# Autodesk Inventor assembly: Frame Assembly
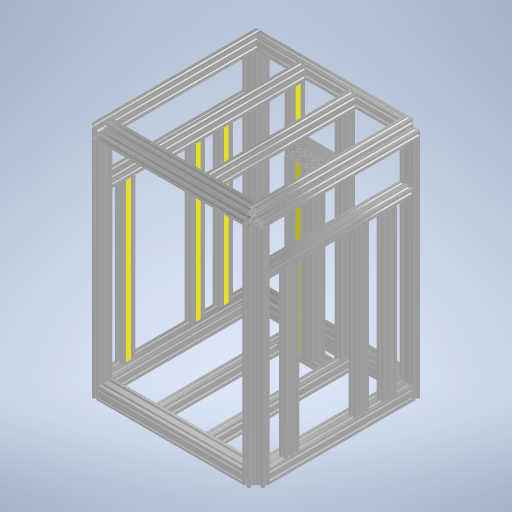
[picture p0: Inventor's stored thumbnail of the model, 512x512]
Saved by Autodesk Inventor 2024 (Build 280153000, 153)
## iProperties
Created: 2024-12-10
Part Number: Frame Assembly
Document SubType Name: Assembly
Designer: Ishaan
Author: Ishaan
## Documents named in this file (27)
- E:\Projects\Axiom--IDEX-3D-Printer\CAD\01 - Frame\Frame Assembly.iam
- E:\Projects\Axiom--IDEX-3D-Printer\CAD\01 - Frame\4040 Back Left Corner.ipt
- E:\Projects\Axiom--IDEX-3D-Printer\CAD\01 - Frame\4040 Back Right Corner.ipt
- E:\Projects\Axiom--IDEX-3D-Printer\CAD\01 - Frame\4040 Front Left Corner.ipt
- E:\Projects\Axiom--IDEX-3D-Printer\CAD\01 - Frame\4040 Front Right Corner.ipt
- E:\Projects\Axiom--IDEX-3D-Printer\CAD\01 - Frame\Front Base Beam.ipt
- E:\Projects\Axiom--IDEX-3D-Printer\CAD\01 - Frame\Left Base Beam.ipt
- E:\Projects\Axiom--IDEX-3D-Printer\CAD\01 - Frame\Rear Base Beam.ipt
- E:\Projects\Axiom--IDEX-3D-Printer\CAD\01 - Frame\Right Base Beam.ipt
- E:\Projects\Axiom--IDEX-3D-Printer\CAD\01 - Frame\2040 Side Anterior Riser.ipt
- E:\Projects\Axiom--IDEX-3D-Printer\CAD\01 - Frame\2040 Side Posterior Riser.ipt
- E:\Projects\Axiom--IDEX-3D-Printer\CAD\01 - Frame\2040 Side Medial Riser.ipt
- E:\Projects\Axiom--IDEX-3D-Printer\CAD\01 - Frame\2040 Left Gantry Extrusion.ipt
- E:\Projects\Axiom--IDEX-3D-Printer\CAD\01 - Frame\2040 Right Gantry Extrusion.ipt
- E:\Projects\Axiom--IDEX-3D-Printer\CAD\01 - Frame\2040 Bottom Left Reinforcement.ipt
- E:\Projects\Axiom--IDEX-3D-Printer\CAD\01 - Frame\2040 Bottom Right Reinforcement.ipt
- E:\Projects\Axiom--IDEX-3D-Printer\CAD\01 - Frame\4040 Top Left Edge.ipt
- E:\Projects\Axiom--IDEX-3D-Printer\CAD\01 - Frame\4040 Top Right Edge.ipt
- E:\Projects\Axiom--IDEX-3D-Printer\CAD\01 - Frame\4040 Top Front Edge.ipt
- E:\Projects\Axiom--IDEX-3D-Printer\CAD\01 - Frame\4040 Top Rear Edge.ipt
- E:\Projects\Axiom--IDEX-3D-Printer\CAD\01 - Frame\2040 Top Left Reinforcement.ipt
- E:\Projects\Axiom--IDEX-3D-Printer\CAD\01 - Frame\2040 Top Right Reinforcement.ipt
- E:\Projects\Axiom--IDEX-3D-Printer\CAD\01 - Frame\2040 Rear Left Riser.ipt
- E:\Projects\Axiom--IDEX-3D-Printer\CAD\01 - Frame\2040 Rear Right Riser.ipt
- E:\Projects\Axiom--IDEX-3D-Printer\CAD\01 - Frame\2040 Z-Rail Brace.ipt
- E:\Projects\Axiom--IDEX-3D-Printer\CAD\01 - Frame\2040 Z-column Support.ipt
- E:\Projects\Axiom--IDEX-3D-Printer\CAD\01 - Frame\4080 Z-rail.ipt
## Components (29 placed, 26 different names)
1. 4040 Back Left Corner:1 — Flush:11, Mate:7, Flush:12, Mate:9, Flush:14, Mate:17
2. 4040 Back Right Corner:1 — Flush:3, Mate:3, Flush:4, Mate:8, Mate:15
3. 4040 Front Left Corner:1 — Flush:7, Mate:5, Flush:8, Mate:6, Flush:9, Flush:10, Flush:16, Mate:13, Mate:23, Mate:30, Flush:25, Flush:26
4. 4040 Front Right Corner:1 — Flush:1, Mate:2, Flush:2, Mate:4, Flush:6, Mate:11, Mate:25, Flush:27, Mate:31, Flush:28
5. Front Base Beam:1 — Flush:5, Mate:4, Flush:6, Flush:7, Mate:5, Flush:8, Mate:26, Flush:23, Mate:28, Flush:24
6. Left Base Beam:1 — Mate:6, Flush:9, Flush:10, Flush:11, Mate:7, Flush:12, Mate:12, Flush:18, Mate:16, Mate:20, Flush:20, Mate:27
7. Rear Base Beam:1 — Flush:13, Mate:8, Mate:9, Flush:14
8. Right Base Beam:1 — Mate:1, Flush:1, Mate:2, Flush:2, Flush:3, Mate:3, Flush:4, Flush:5, Flush:13, Mate:10, Flush:15, Mate:14, Flush:17, Mate:18, Flush:19, Mate:29
9. 2040 Side Anterior Riser:1 — Mate:10, Flush:15, Mate:11, Mate:19, Flush:22
10. 2040 Side Anterior Riser:2 — Mate:12, Flush:16, Mate:13, Mate:21
11. 2040 Side Posterior Riser:1 — Mate:14, Flush:17, Mate:15, Mate:24, Mate:43
12. 2040 Side Posterior Riser:2 — Flush:18, Mate:16, Mate:17, Flush:42
13. 2040 Side Medial Riser:1 — Mate:18, Flush:19, Mate:19
14. 2040 Side Medial Riser:2 — Mate:20, Flush:20, Mate:21, Mate:22, Flush:21
15. 2040 Left Gantry Extrusion:1 — Mate:22, Mate:23, Flush:21
16. 2040 Right Gantry Extrusion:1 — Mate:24, Mate:25, Flush:22
17. 2040 Bottom Left Reinforcement:1 — Mate:28, Flush:24, Mate:29, Mate:40, Flush:33, Mate:48
18. 2040 Bottom Right Reinforcement:1 — Mate:26, Flush:23, Mate:27, Mate:42, Flush:34, Flush:41
19. 4040 Top Left Edge:1 — Flush:27, Mate:31, Flush:28, Mate:39
20. 4040 Top Right Edge:1 — Mate:30, Flush:25, Flush:26, Mate:37
21. 4040 Top Rear Edge:1
22. 4040 Top Front Edge:2 — Mate:36, Flush:31, Mate:38, Flush:32
23. 2040 Top Left Reinforcement:1 — Mate:38, Flush:32, Mate:39
24. 2040 Top Right Reinforcement:1 — Mate:36, Flush:31, Mate:37
25. 2040 Rear Left Riser:1 — Mate:42, Flush:34, Flush:35, Mate:47, Flush:40, Mate:50
26. 2040 Rear Right Riser:1 — Mate:40, Flush:33, Flush:35, Mate:43
27. 2040 Z-Rail Brace:1 — Mate:47, Flush:40, Flush:44
28. 2040 Z-column Support:1 — Flush:41, Mate:48, Flush:42, Mate:49, Flush:43
29. 4080 Z-rail:1 — Mate:49, Flush:43, Mate:50, Flush:44
## Relationships (86: Mate 46, Flush 40)
- Mate:1: Right Base Beam:1
- Flush:1: 4040 Front Right Corner:1 ↔ Right Base Beam:1
- Mate:2: 4040 Front Right Corner:1 ↔ Right Base Beam:1
- Flush:2: 4040 Front Right Corner:1 ↔ Right Base Beam:1
- Flush:3: 4040 Back Right Corner:1 ↔ Right Base Beam:1
- Mate:3: 4040 Back Right Corner:1 ↔ Right Base Beam:1
- Flush:4: 4040 Back Right Corner:1 ↔ Right Base Beam:1
- Flush:5: Front Base Beam:1 ↔ Right Base Beam:1
- Mate:4: 4040 Front Right Corner:1 ↔ Front Base Beam:1
- Flush:6: 4040 Front Right Corner:1 ↔ Front Base Beam:1
- Flush:7: 4040 Front Left Corner:1 ↔ Front Base Beam:1
- Mate:5: 4040 Front Left Corner:1 ↔ Front Base Beam:1
- Flush:8: 4040 Front Left Corner:1 ↔ Front Base Beam:1
- Mate:6: 4040 Front Left Corner:1 ↔ Left Base Beam:1
- Flush:9: 4040 Front Left Corner:1 ↔ Left Base Beam:1
- Flush:10: 4040 Front Left Corner:1 ↔ Left Base Beam:1
- Flush:11: 4040 Back Left Corner:1 ↔ Left Base Beam:1
- Mate:7: 4040 Back Left Corner:1 ↔ Left Base Beam:1
- Flush:12: 4040 Back Left Corner:1 ↔ Left Base Beam:1
- Flush:13: Rear Base Beam:1 ↔ Right Base Beam:1
- Mate:8: 4040 Back Right Corner:1 ↔ Rear Base Beam:1
- Mate:9: 4040 Back Left Corner:1 ↔ Rear Base Beam:1
- Flush:14: 4040 Back Left Corner:1 ↔ Rear Base Beam:1
- Mate:10: Right Base Beam:1 ↔ 2040 Side Anterior Riser:1
- Flush:15: Right Base Beam:1 ↔ 2040 Side Anterior Riser:1
- Mate:11 (46 mm): 4040 Front Right Corner:1 ↔ 2040 Side Anterior Riser:1
- Mate:12: Left Base Beam:1 ↔ 2040 Side Anterior Riser:2
- Flush:16: 4040 Front Left Corner:1 ↔ 2040 Side Anterior Riser:2
- Mate:13 (46 mm): 4040 Front Left Corner:1 ↔ 2040 Side Anterior Riser:2
- Mate:14: Right Base Beam:1 ↔ 2040 Side Posterior Riser:1
- Flush:17: Right Base Beam:1 ↔ 2040 Side Posterior Riser:1
- Mate:15 (46 mm): 4040 Back Right Corner:1 ↔ 2040 Side Posterior Riser:1
- Flush:18: Left Base Beam:1 ↔ 2040 Side Posterior Riser:2
- Mate:16: Left Base Beam:1 ↔ 2040 Side Posterior Riser:2
- Mate:17 (46 mm): 4040 Back Left Corner:1 ↔ 2040 Side Posterior Riser:2
- Mate:18: Right Base Beam:1 ↔ 2040 Side Medial Riser:1
- Flush:19: Right Base Beam:1 ↔ 2040 Side Medial Riser:1
- Mate:19 (162 mm): 2040 Side Anterior Riser:1 ↔ 2040 Side Medial Riser:1
- Mate:20: Left Base Beam:1 ↔ 2040 Side Medial Riser:2
- Flush:20: Left Base Beam:1 ↔ 2040 Side Medial Riser:2
- Mate:21 (162 mm): 2040 Side Anterior Riser:2 ↔ 2040 Side Medial Riser:2
- Mate:22: 2040 Side Medial Riser:2 ↔ 2040 Left Gantry Extrusion:1
- Mate:23: 4040 Front Left Corner:1 ↔ 2040 Left Gantry Extrusion:1
- Flush:21: 2040 Side Medial Riser:2 ↔ 2040 Left Gantry Extrusion:1
- Mate:24: 2040 Side Posterior Riser:1 ↔ 2040 Right Gantry Extrusion:1
- Mate:25: 4040 Front Right Corner:1 ↔ 2040 Right Gantry Extrusion:1
- Flush:22: 2040 Side Anterior Riser:1 ↔ 2040 Right Gantry Extrusion:1
- Mate:26: Front Base Beam:1 ↔ 2040 Bottom Right Reinforcement:1
- Flush:23: Front Base Beam:1 ↔ 2040 Bottom Right Reinforcement:1
- Mate:27 (125 mm): Left Base Beam:1 ↔ 2040 Bottom Right Reinforcement:1
- Mate:28: Front Base Beam:1 ↔ 2040 Bottom Left Reinforcement:1
- Flush:24: Front Base Beam:1 ↔ 2040 Bottom Left Reinforcement:1
- Mate:29 (125 mm): Right Base Beam:1 ↔ 2040 Bottom Left Reinforcement:1
- Mate:30: 4040 Front Left Corner:1 ↔ 4040 Top Right Edge:1
- Flush:25: 4040 Front Left Corner:1 ↔ 4040 Top Right Edge:1
- Flush:26: 4040 Front Left Corner:1 ↔ 4040 Top Right Edge:1
- Flush:27: 4040 Front Right Corner:1 ↔ 4040 Top Left Edge:1
- Mate:31: 4040 Front Right Corner:1 ↔ 4040 Top Left Edge:1
- Flush:28: 4040 Front Right Corner:1 ↔ 4040 Top Left Edge:1
- [Mate]: 4040 Front Left Corner:1 ↔ 4040 Top Front Edge:2
- [Mate]: 4040 Front Right Corner:1 ↔ 4040 Top Front Edge:2
- [Flush]: 4040 Top Right Edge:1 ↔ 4040 Top Front Edge:2
- [Mate]: 4040 Back Left Corner:1 ↔ 4040 Top Rear Edge:1
- [Mate]: 4040 Top Left Edge:1 ↔ 4040 Top Rear Edge:1
- [Flush]: 4040 Back Left Corner:1 ↔ 4040 Top Rear Edge:1
- Mate:36: 4040 Top Front Edge:2 ↔ 2040 Top Right Reinforcement:1
- Flush:31: 4040 Top Front Edge:2 ↔ 2040 Top Right Reinforcement:1
- Mate:37 (125 mm): 4040 Top Right Edge:1 ↔ 2040 Top Right Reinforcement:1
- Mate:38: 4040 Top Front Edge:2 ↔ 2040 Top Left Reinforcement:1
- Flush:32: 4040 Top Front Edge:2 ↔ 2040 Top Left Reinforcement:1
- Mate:39 (125 mm): 4040 Top Left Edge:1 ↔ 2040 Top Left Reinforcement:1
- Mate:40: 2040 Bottom Left Reinforcement:1 ↔ 2040 Rear Right Riser:1
- Flush:33: 2040 Bottom Left Reinforcement:1 ↔ 2040 Rear Right Riser:1
- Mate:42: 2040 Bottom Right Reinforcement:1 ↔ 2040 Rear Left Riser:1
- Flush:34: 2040 Bottom Right Reinforcement:1 ↔ 2040 Rear Left Riser:1
- Flush:35: 2040 Rear Left Riser:1 ↔ 2040 Rear Right Riser:1
- Mate:43 (3 mm): 2040 Side Posterior Riser:1 ↔ 2040 Rear Right Riser:1
- Mate:47: 2040 Rear Left Riser:1 ↔ 2040 Z-Rail Brace:1
- Flush:40: 2040 Rear Left Riser:1 ↔ 2040 Z-Rail Brace:1
- Flush:41: 2040 Bottom Right Reinforcement:1 ↔ 2040 Z-column Support:1
- Mate:48: 2040 Bottom Left Reinforcement:1 ↔ 2040 Z-column Support:1
- Flush:42: 2040 Side Posterior Riser:2 ↔ 2040 Z-column Support:1
- Mate:49: 2040 Z-column Support:1 ↔ 4080 Z-rail:1
- Flush:43: 2040 Z-column Support:1 ↔ 4080 Z-rail:1
- Mate:50 (22.5 mm): 2040 Rear Left Riser:1 ↔ 4080 Z-rail:1
- Flush:44: 2040 Z-Rail Brace:1 ↔ 4080 Z-rail:1
